# Autodesk Inventor assembly: case_asm
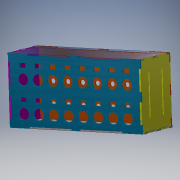
[picture p0: Inventor's stored thumbnail of the model, 180x180]
Saved by Autodesk Inventor 2019 (Build 230136000, 136)
## iProperties
Created: 2019-07-12
Part Number: case_asm
Document SubType Name: Assembly
Designer: Lino P
Author: Lino P
## Documents named in this file (5)
- C:\Users\Lino P\Documents\000 - USFQ\TesisDev\ipt\case_asm.iam
- C:\Users\Lino P\Documents\000 - USFQ\TesisDev\ipt\case_back.ipt
- C:\Users\Lino P\Documents\000 - USFQ\TesisDev\ipt\case_front.ipt
- C:\Users\Lino P\Documents\000 - USFQ\TesisDev\ipt\case_side.ipt
- C:\Users\Lino P\Documents\000 - USFQ\TesisDev\ipt\case_roof.ipt
## Components (6 placed, 4 different names)
1. case_back:1 — Mate:4, Mate:5, Mate:6, Mate:7
2. case_front:1 — Mate:1, Mate:2, Mate:3, Mate:8, Mate:9, Mate:10, Mate:11, Mate:12, Mate:13, Mate:14, Mate:15, Mate:16
3. case_side:1 — Mate:8, Mate:9, Mate:10
4. case_side:2 — Mate:1, Mate:2, Mate:3, Mate:4, Mate:5, Mate:6
5. case_roof:1 — Mate:11, Mate:12, Mate:13
6. case_roof:2 — Mate:14, Mate:15, Mate:16
## Relationships (16: Mate 16)
- Mate:1: case_front:1 ↔ case_side:2
- Mate:2: case_front:1 ↔ case_side:2
- Mate:3: case_front:1 ↔ case_side:2
- Mate:4: case_back:1 ↔ case_side:2
- Mate:5: case_back:1 ↔ case_side:2
- Mate:6: case_back:1 ↔ case_side:2
- Mate:7: case_back:1
- Mate:8: case_front:1 ↔ case_side:1
- Mate:9: case_front:1 ↔ case_side:1
- Mate:10: case_front:1 ↔ case_side:1
- Mate:11: case_front:1 ↔ case_roof:1
- Mate:12: case_front:1 ↔ case_roof:1
- Mate:13: case_front:1 ↔ case_roof:1
- Mate:14: case_front:1 ↔ case_roof:2
- Mate:15: case_front:1 ↔ case_roof:2
- Mate:16: case_front:1 ↔ case_roof:2
